# Autodesk Inventor assembly: My_Pen_Case_4pens
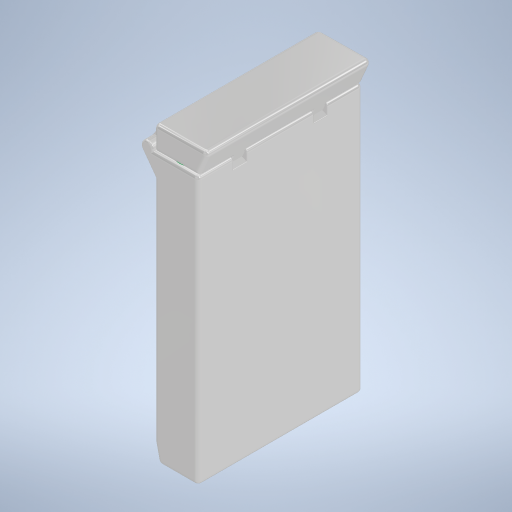
[picture p0: Inventor's stored thumbnail of the model, 512x512]
Saved by Autodesk Inventor 2024 (Build 280153000, 153)
## iProperties
Created: 2024-12-19
Part Number: My_Pen_Case_4pens
Document SubType Name: Assembly
Designer: Emil
Author: Emil
## Documents named in this file (3)
- C:\Users\Emil\OneDrive\Dokument\Projekt-Emil\Fountain_pen+Case+Pen_Holder\InventorCad\My_Pen_Cases\My_Pen_Case_4pens\My_Pen_Case_4pens.iam
- C:\Users\Emil\OneDrive\Dokument\Projekt-Emil\Fountain_pen+Case+Pen_Holder\InventorCad\My_Pen_Cases\My_Pen_Case_4pens\Body_4pens.ipt
- C:\Users\Emil\OneDrive\Dokument\Projekt-Emil\Fountain_pen+Case+Pen_Holder\InventorCad\My_Pen_Cases\My_Pen_Case_4pens\Lid_4pens.ipt
## Components (2 placed, 2 different names)
1. Body_4pens:1 — Insert:1
2. Lid_4pens:1 — Insert:1
## Relationships (1: Insert 1)
- Insert:1 (0.2 mm): Body_4pens:1 ↔ Lid_4pens:1
